# Autodesk Inventor assembly: Dual Extruder With Auto Leveling
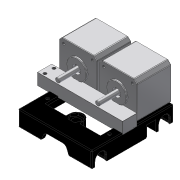
[picture p0: Inventor's stored thumbnail of the model, 180x180]
Saved by Autodesk Inventor 2015 (Build 190159000, 159)
## iProperties
Created: 2020-01-08
Part Number: Dual Extruder With Auto Leveling
Document SubType Name: Assembly
Designer: Ghassan Yusuf
Author: Ghassan Yusuf
## Documents named in this file (5)
- D:\Dropbox\Autodesk Designs\MakerBot Transformation\Dual Extruder With Auto Leveling.iam
- D:\Dropbox\Autodesk Designs\MakerBot Transformation\Stepper Motor.ipt
- C:\Users\Ghassan Yusuf\Dropbox\Autodesk Designs\Filament-Press.ipt
- D:\Dropbox\Autodesk Designs\MakerBot Transformation\Aluminum Mounting Bridge.ipt
- D:\Dropbox\Autodesk Designs\MakerBot Transformation\Carriage.ipt
## Components (5 placed, 4 different names)
1. Stepper Motor:1 — Mate:1, Flush:1, Flush:2, Mate:2, Flush:3, Flush:7
2. Filament-Press:1
3. Aluminum Mounting Bridge:1 — Mate:2, Flush:3, Mate:5, Flush:6, Mate:6, Flush:7
4. Stepper Motor:2 — Mate:1, Flush:1, Flush:2
5. Carriage:1 — Mate:5, Flush:6, Mate:6
## Relationships (9: Flush 5, Mate 4)
- Mate:1 (2 mm): Stepper Motor:1 ↔ Stepper Motor:2
- Flush:1: Stepper Motor:1 ↔ Stepper Motor:2
- Flush:2: Stepper Motor:1 ↔ Stepper Motor:2
- Mate:2: Stepper Motor:1 ↔ Aluminum Mounting Bridge:1
- Flush:3: Stepper Motor:1 ↔ Aluminum Mounting Bridge:1
- Mate:5: Aluminum Mounting Bridge:1 ↔ Carriage:1
- Flush:6: Aluminum Mounting Bridge:1 ↔ Carriage:1
- Mate:6: Aluminum Mounting Bridge:1 ↔ Carriage:1
- Flush:7: Stepper Motor:1 ↔ Aluminum Mounting Bridge:1
